# Autodesk Inventor assembly: AssemblyV1
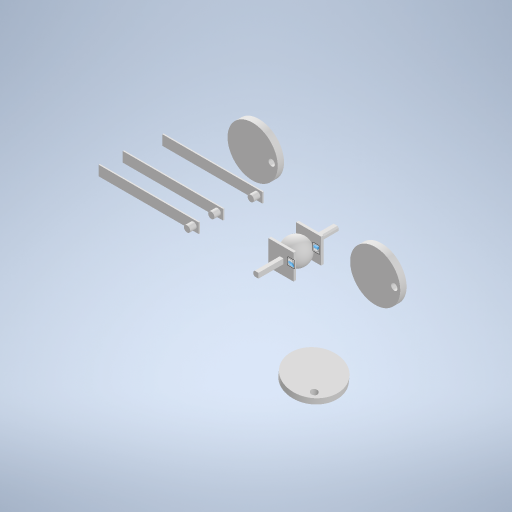
[picture p0: Inventor's stored thumbnail of the model, 512x512]
Saved by Autodesk Inventor 2024 (Build 280153000, 153)
## iProperties
Created: 2024-01-14
Part Number: AssemblyV1
Document SubType Name: Assembly
Designer: Owner
Author: Owner
## Documents named in this file (5)
- C:\Users\Owner\PycharmProjects\DodgeBot\CAD_FILES\AssemblyV1.iam
- C:\Users\Owner\PycharmProjects\DodgeBot\CAD_FILES\Ball Joint.ipt
- C:\Users\Owner\PycharmProjects\DodgeBot\CAD_FILES\Post.ipt
- C:\Users\Owner\PycharmProjects\DodgeBot\CAD_FILES\Belt.ipt
- C:\Users\Owner\PycharmProjects\DodgeBot\CAD_FILES\Wheel_Consept.ipt
## Components (9 placed, 4 different names)
1. Ball Joint:1 — Rigid:1, Rigid:2
2. Post:1 — Rigid:1
3. Post:2 — Rigid:2
4. Belt:1
5. Belt:2
6. Belt:3
7. Wheel_Consept:1
8. Wheel_Consept:2
9. Wheel_Consept:3
## Relationships (2: WeldJoint 2)
- Rigid:1 [WeldJoint] (250 mm): Ball Joint:1 ↔ Post:1
- Rigid:2 [WeldJoint] (-250 mm): Ball Joint:1 ↔ Post:2
